# Autodesk Inventor assembly: BeamAssembly
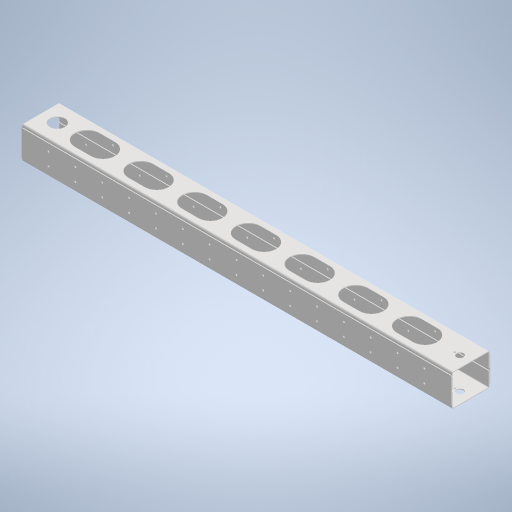
[picture p0: Inventor's stored thumbnail of the model, 512x512]
Saved by Autodesk Inventor 2023 (Build 270158000, 158)
## iProperties
Created: 2023-05-02
Part Number: BeamAssembly
Document SubType Name: Assembly
Designer: emila
Author: emila
## Documents named in this file (3)
- C:\Users\emila\Documents\Inventor\BeamAssembly.iam
- C:\Users\emila\Documents\Inventor\beam.ipt
- C:\Users\emila\Documents\Inventor\connectionPlate.ipt
## Components (4 placed, 2 different names)
1. beam:1 — Flush:1, Flush:2, Mate:5
2. beam:2 — Flush:1, Flush:2, Mate:1, Mate:2, Mate:3, Mate:4
3. connectionPlate:1 — Mate:1, Mate:3, Mate:5
4. connectionPlate:2 — Mate:2, Mate:4
## Relationships (7: Mate 5, Flush 2)
- Flush:1: beam:1 ↔ beam:2
- Flush:2: beam:1 ↔ beam:2
- Mate:1: beam:2 ↔ connectionPlate:1
- Mate:2: beam:2 ↔ connectionPlate:2
- Mate:3: beam:2 ↔ connectionPlate:1
- Mate:4: beam:2 ↔ connectionPlate:2
- Mate:5: beam:1 ↔ connectionPlate:1
